# Autodesk Inventor assembly: Timing_Assy_Star Shaft 3 Lanes
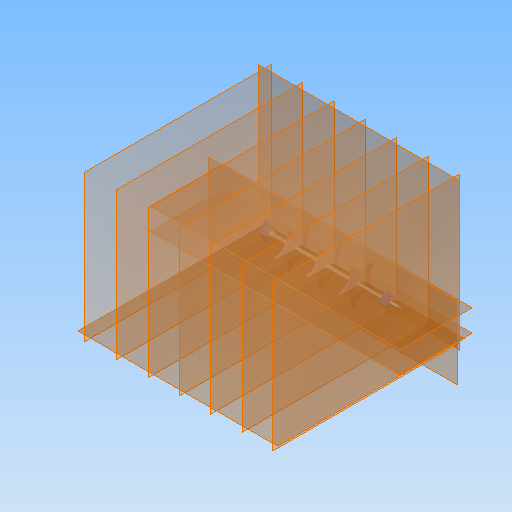
[picture p0: Inventor's stored thumbnail of the model, 512x512]
Saved by Autodesk Inventor 2018.1 (Build 221171000, 171)
## iProperties
Created: 2019-02-11
Part Number: Timing_Assy_Star Shaft 3 Lanes
Document SubType Name: Assembly
Designer: James
Mass: 92.827 g
Surface Area: 261.339 cm^2
Volume: 33.0472 cm^3
Density: 2.80892 g/cm^3
Author: James
## Documents named in this file (5)
- C:\Users\admin\Desktop\Ball-Machine\Timing Gate\Timing - 3 Lanes\Timing_Assy_Star Shaft 3 Lanes.iam
- C:\Users\admin\Desktop\Ball-Machine\Timing Gate\Timing_Star.ipt
- C:\Users\admin\Desktop\Ball-Machine\Timing Gate\BS 3673 - 6mm External Circlip.ipt
- C:\Users\admin\Desktop\Ball-Machine\Timing Gate\SAFL212 Oval 2 Bolt Flanged Unit.ipt
- C:\Users\admin\Desktop\Ball-Machine\Timing Gate\Timing - 3 Lanes\Timing_Star Shaft 3 Lanes.ipt
## Components (11 placed, 4 different names)
1. Timing_Star Shaft 3 Lanes:1 — Mate:4, Flush:6, Flush:14, Flush:15, Mate:49, Mate:50, Angle:3, Mate:61, Mate:62, Mate:63, Mate:66, Flush:28, Mate:68
2. SAFL212 Oval 2 Bolt Flanged Unit:1 — Mate:61, Flush:24, Angle:4, Mate:65
3. SAFL212 Oval 2 Bolt Flanged Unit:2 — Mate:62, Flush:24, Mate:64, Mate:67
4. BS 3673 - 6mm External Circlip:16 — Mate:65, Mate:66, Flush:25, Mate:68
5. BS 3673 - 6mm External Circlip:17 — Mate:63, Mate:64, Flush:25, Flush:26
6. BS 3673 - 6mm External Circlip:11 — Mate:49, Mate:50, Angle:3, Flush:26
7. Timing_Star:1 — Mate:4, Flush:28
8. BS 3673 - 6mm External Circlip:12
9. Timing_Star:2
10. BS 3673 - 6mm External Circlip:13
11. Timing_Star:3
## Component patterns: (3 elements, first: BS 3673 - 6mm External Circlip:11 + Timing_Star:1)
## Relationships (23: Mate 11, Flush 10, Angle 2)
- Mate:4: Timing_Star Shaft 3 Lanes:1 ↔ Timing_Star:1
- Flush:6: Timing_Star Shaft 3 Lanes:1
- Flush:11 (-58 mm)
- Flush:12 (-5 mm)
- Flush:13 (30 mm)
- Flush:14: Timing_Star Shaft 3 Lanes:1
- Flush:15: Timing_Star Shaft 3 Lanes:1
- Mate:49: Timing_Star Shaft 3 Lanes:1 ↔ BS 3673 - 6mm External Circlip:11
- Mate:50: Timing_Star Shaft 3 Lanes:1 ↔ BS 3673 - 6mm External Circlip:11
- Angle:3 (0 deg): Timing_Star Shaft 3 Lanes:1 ↔ BS 3673 - 6mm External Circlip:11
- Mate:61: Timing_Star Shaft 3 Lanes:1 ↔ SAFL212 Oval 2 Bolt Flanged Unit:1
- Mate:62: Timing_Star Shaft 3 Lanes:1 ↔ SAFL212 Oval 2 Bolt Flanged Unit:2
- Flush:24: SAFL212 Oval 2 Bolt Flanged Unit:1 ↔ SAFL212 Oval 2 Bolt Flanged Unit:2
- Angle:4 (0 deg): SAFL212 Oval 2 Bolt Flanged Unit:1
- Mate:63: Timing_Star Shaft 3 Lanes:1 ↔ BS 3673 - 6mm External Circlip:17
- Mate:64: SAFL212 Oval 2 Bolt Flanged Unit:2 ↔ BS 3673 - 6mm External Circlip:17
- Mate:65: SAFL212 Oval 2 Bolt Flanged Unit:1 ↔ BS 3673 - 6mm External Circlip:16
- Mate:66: Timing_Star Shaft 3 Lanes:1 ↔ BS 3673 - 6mm External Circlip:16
- Flush:25: BS 3673 - 6mm External Circlip:16 ↔ BS 3673 - 6mm External Circlip:17
- Flush:26: BS 3673 - 6mm External Circlip:17 ↔ BS 3673 - 6mm External Circlip:11
- Mate:67: SAFL212 Oval 2 Bolt Flanged Unit:2
- Flush:28: Timing_Star Shaft 3 Lanes:1 ↔ Timing_Star:1
- Mate:68: Timing_Star Shaft 3 Lanes:1 ↔ BS 3673 - 6mm External Circlip:16
